# Autodesk Inventor assembly: CardGuideArray-Long
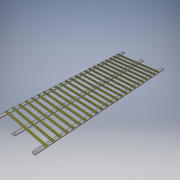
[picture p0: Inventor's stored thumbnail of the model, 180x180]
Saved by Autodesk Inventor 2018 (Build 220112000, 112)
## iProperties
Created: 2025-02-19
Part Number: CardGuideArray-Long
Material: Všeobecné
Document SubType Name: Assembly
Designer: Jozko Mrkvicka
Author: Jozko Mrkvicka
## Documents named in this file (5)
- D:\05_Projekty\Projects_Inventor\Haluska9000\CardGuideArray-8-Inch.iam
- D:\05_Projekty\Projects_Inventor\Haluska9000\CardGuide.ipt
- D:\05_Projekty\Projects_Inventor\Haluska9000\Profile-Flat.ipt
- D:\05_Projekty\Projects_Inventor\Haluska9000\Profile-Flat\Profile-Flat#Cabinet-FerriteCore-Width.ipt
- D:\05_Projekty\Projects_Inventor\Haluska9000\CardGuide\CardGuide#8-inch.ipt
## Components (26 placed, 2 different names)
1. Profile-Flat#Cabinet-FerriteCore-Width:3 — Stejný směr:3, Stejný směr:4, Proti sobě:93, Proti sobě:94, Proti sobě:95, Proti sobě:96, Proti sobě:97, Proti sobě:98, Proti sobě:99, Proti sobě:100, Proti sobě:101, Proti sobě:102, Proti sobě:114, Proti sobě:115, Proti sobě:116, Proti sobě:117, Proti sobě:118, Proti sobě:119, Proti sobě:120, Proti sobě:121, Proti sobě:122, Proti sobě:123, Proti sobě:124, Proti sobě:125, Proti sobě:126, Proti sobě:127, Proti sobě:128, Proti sobě:129, Proti sobě:130, Proti sobě:131, Proti sobě:132, Proti sobě:133, Proti sobě:134, Proti sobě:135, Proti sobě:136
2. Profile-Flat#Cabinet-FerriteCore-Width:4 — Proti sobě:42, Proti sobě:43, Proti sobě:44, Proti sobě:45, Proti sobě:46, Proti sobě:47, Proti sobě:48, Proti sobě:49, Proti sobě:50, Proti sobě:51, Proti sobě:52, Proti sobě:53, Proti sobě:54, Proti sobě:55, Proti sobě:56, Proti sobě:57, Proti sobě:58, Proti sobě:59, Proti sobě:60, Proti sobě:61, Proti sobě:62, Proti sobě:63, Proti sobě:64, Proti sobě:65, Proti sobě:66, Proti sobě:67, Stejný směr:3, Stejný směr:4, Stejný směr:5, Proti sobě:103, Proti sobě:104, Proti sobě:105, Proti sobě:106, Proti sobě:107, Proti sobě:108, Proti sobě:109, Proti sobě:110, Proti sobě:111, Proti sobě:112, Proti sobě:113
3. Profile-Flat#Cabinet-FerriteCore-Width:5 — Stejný směr:5
4. CardGuide#8-inch:14 — Proti sobě:45, Proti sobě:64, Proti sobě:129
5. CardGuide#8-inch:15 — Proti sobě:46, Proti sobě:63, Proti sobě:128
6. CardGuide#8-inch:16 — Proti sobě:54, Proti sobě:55, Proti sobě:119
7. CardGuide#8-inch:17 — Proti sobě:44, Proti sobě:65, Proti sobě:130
8. CardGuide#8-inch:18 — Proti sobě:47, Proti sobě:62, Proti sobě:127
9. CardGuide#8-inch:19 — Proti sobě:48, Proti sobě:61, Proti sobě:126
10. CardGuide#8-inch:20 — Proti sobě:42, Proti sobě:67, Proti sobě:120
11. CardGuide#8-inch:21 — Proti sobě:43, Proti sobě:66, Proti sobě:131
12. CardGuide#8-inch:22 — Proti sobě:50, Proti sobě:59, Proti sobě:124
13. CardGuide#8-inch:23 — Proti sobě:51, Proti sobě:58, Proti sobě:123
14. CardGuide#8-inch:24 — Proti sobě:52, Proti sobě:57, Proti sobě:122
15. CardGuide#8-inch:25 — Proti sobě:53, Proti sobě:56, Proti sobě:121
16. CardGuide#8-inch:26 — Proti sobě:49, Proti sobě:60, Proti sobě:125
17. CardGuide#8-inch:27 — Proti sobě:95, Proti sobě:105, Proti sobě:134
18. CardGuide#8-inch:28 — Proti sobě:96, Proti sobě:104, Proti sobě:133
19. CardGuide#8-inch:29 — Proti sobě:94, Proti sobě:106, Proti sobě:135
20. CardGuide#8-inch:30 — Proti sobě:97, Proti sobě:103, Proti sobě:132
21. CardGuide#8-inch:31 — Proti sobě:93, Proti sobě:107, Proti sobě:136
22. CardGuide#8-inch:32 — Proti sobě:100, Proti sobě:110, Proti sobě:116
23. CardGuide#8-inch:33 — Proti sobě:101, Proti sobě:111, Proti sobě:115
24. CardGuide#8-inch:34 — Proti sobě:99, Proti sobě:109, Proti sobě:117
25. CardGuide#8-inch:35 — Proti sobě:102, Proti sobě:112, Proti sobě:114
26. CardGuide#8-inch:36 — Proti sobě:98, Proti sobě:108, Proti sobě:118
## Relationships (73: Mate 70, Flush 3)
- Proti sobě:42 [Mate]: Profile-Flat#Cabinet-FerriteCore-Width:4 ↔ CardGuide#8-inch:20
- Proti sobě:43 [Mate]: Profile-Flat#Cabinet-FerriteCore-Width:4 ↔ CardGuide#8-inch:21
- Proti sobě:44 [Mate]: Profile-Flat#Cabinet-FerriteCore-Width:4 ↔ CardGuide#8-inch:17
- Proti sobě:45 [Mate]: Profile-Flat#Cabinet-FerriteCore-Width:4 ↔ CardGuide#8-inch:14
- Proti sobě:46 [Mate]: Profile-Flat#Cabinet-FerriteCore-Width:4 ↔ CardGuide#8-inch:15
- Proti sobě:47 [Mate]: Profile-Flat#Cabinet-FerriteCore-Width:4 ↔ CardGuide#8-inch:18
- Proti sobě:48 [Mate]: Profile-Flat#Cabinet-FerriteCore-Width:4 ↔ CardGuide#8-inch:19
- Proti sobě:49 [Mate]: Profile-Flat#Cabinet-FerriteCore-Width:4 ↔ CardGuide#8-inch:26
- Proti sobě:50 [Mate]: Profile-Flat#Cabinet-FerriteCore-Width:4 ↔ CardGuide#8-inch:22
- Proti sobě:51 [Mate]: Profile-Flat#Cabinet-FerriteCore-Width:4 ↔ CardGuide#8-inch:23
- Proti sobě:52 [Mate]: Profile-Flat#Cabinet-FerriteCore-Width:4 ↔ CardGuide#8-inch:24
- Proti sobě:53 [Mate]: Profile-Flat#Cabinet-FerriteCore-Width:4 ↔ CardGuide#8-inch:25
- Proti sobě:54 [Mate]: Profile-Flat#Cabinet-FerriteCore-Width:4 ↔ CardGuide#8-inch:16
- Proti sobě:55 [Mate]: Profile-Flat#Cabinet-FerriteCore-Width:4 ↔ CardGuide#8-inch:16
- Proti sobě:56 [Mate]: Profile-Flat#Cabinet-FerriteCore-Width:4 ↔ CardGuide#8-inch:25
- Proti sobě:57 [Mate]: Profile-Flat#Cabinet-FerriteCore-Width:4 ↔ CardGuide#8-inch:24
- Proti sobě:58 [Mate]: Profile-Flat#Cabinet-FerriteCore-Width:4 ↔ CardGuide#8-inch:23
- Proti sobě:59 [Mate]: Profile-Flat#Cabinet-FerriteCore-Width:4 ↔ CardGuide#8-inch:22
- Proti sobě:60 [Mate]: Profile-Flat#Cabinet-FerriteCore-Width:4 ↔ CardGuide#8-inch:26
- Proti sobě:61 [Mate]: Profile-Flat#Cabinet-FerriteCore-Width:4 ↔ CardGuide#8-inch:19
- Proti sobě:62 [Mate]: Profile-Flat#Cabinet-FerriteCore-Width:4 ↔ CardGuide#8-inch:18
- Proti sobě:63 [Mate]: Profile-Flat#Cabinet-FerriteCore-Width:4 ↔ CardGuide#8-inch:15
- Proti sobě:64 [Mate]: Profile-Flat#Cabinet-FerriteCore-Width:4 ↔ CardGuide#8-inch:14
- Proti sobě:65 [Mate]: Profile-Flat#Cabinet-FerriteCore-Width:4 ↔ CardGuide#8-inch:17
- Proti sobě:66 [Mate]: Profile-Flat#Cabinet-FerriteCore-Width:4 ↔ CardGuide#8-inch:21
- Proti sobě:67 [Mate]: Profile-Flat#Cabinet-FerriteCore-Width:4 ↔ CardGuide#8-inch:20
- Stejný směr:3 [Flush]: Profile-Flat#Cabinet-FerriteCore-Width:3 ↔ Profile-Flat#Cabinet-FerriteCore-Width:4
- Stejný směr:4 [Flush]: Profile-Flat#Cabinet-FerriteCore-Width:3 ↔ Profile-Flat#Cabinet-FerriteCore-Width:4
- Stejný směr:5 [Flush]: Profile-Flat#Cabinet-FerriteCore-Width:4 ↔ Profile-Flat#Cabinet-FerriteCore-Width:5
- Proti sobě:93 [Mate]: Profile-Flat#Cabinet-FerriteCore-Width:3 ↔ CardGuide#8-inch:31
- Proti sobě:94 [Mate]: Profile-Flat#Cabinet-FerriteCore-Width:3 ↔ CardGuide#8-inch:29
- Proti sobě:95 [Mate]: Profile-Flat#Cabinet-FerriteCore-Width:3 ↔ CardGuide#8-inch:27
- Proti sobě:96 [Mate]: Profile-Flat#Cabinet-FerriteCore-Width:3 ↔ CardGuide#8-inch:28
- Proti sobě:97 [Mate]: Profile-Flat#Cabinet-FerriteCore-Width:3 ↔ CardGuide#8-inch:30
- Proti sobě:98 [Mate]: Profile-Flat#Cabinet-FerriteCore-Width:3 ↔ CardGuide#8-inch:36
- Proti sobě:99 [Mate]: Profile-Flat#Cabinet-FerriteCore-Width:3 ↔ CardGuide#8-inch:34
- Proti sobě:100 [Mate]: Profile-Flat#Cabinet-FerriteCore-Width:3 ↔ CardGuide#8-inch:32
- Proti sobě:101 [Mate]: Profile-Flat#Cabinet-FerriteCore-Width:3 ↔ CardGuide#8-inch:33
- Proti sobě:102 [Mate]: Profile-Flat#Cabinet-FerriteCore-Width:3 ↔ CardGuide#8-inch:35
- Proti sobě:103 [Mate]: Profile-Flat#Cabinet-FerriteCore-Width:4 ↔ CardGuide#8-inch:30
- Proti sobě:104 [Mate]: Profile-Flat#Cabinet-FerriteCore-Width:4 ↔ CardGuide#8-inch:28
- Proti sobě:105 [Mate]: Profile-Flat#Cabinet-FerriteCore-Width:4 ↔ CardGuide#8-inch:27
- Proti sobě:106 [Mate]: Profile-Flat#Cabinet-FerriteCore-Width:4 ↔ CardGuide#8-inch:29
- Proti sobě:107 [Mate]: Profile-Flat#Cabinet-FerriteCore-Width:4 ↔ CardGuide#8-inch:31
- Proti sobě:108 [Mate]: Profile-Flat#Cabinet-FerriteCore-Width:4 ↔ CardGuide#8-inch:36
- Proti sobě:109 [Mate]: Profile-Flat#Cabinet-FerriteCore-Width:4 ↔ CardGuide#8-inch:34
- Proti sobě:110 [Mate]: Profile-Flat#Cabinet-FerriteCore-Width:4 ↔ CardGuide#8-inch:32
- Proti sobě:111 [Mate]: Profile-Flat#Cabinet-FerriteCore-Width:4 ↔ CardGuide#8-inch:33
- Proti sobě:112 [Mate]: Profile-Flat#Cabinet-FerriteCore-Width:4 ↔ CardGuide#8-inch:35
- Proti sobě:113 [Mate]: Profile-Flat#Cabinet-FerriteCore-Width:4
- Proti sobě:114 [Mate]: Profile-Flat#Cabinet-FerriteCore-Width:3 ↔ CardGuide#8-inch:35
- Proti sobě:115 [Mate]: Profile-Flat#Cabinet-FerriteCore-Width:3 ↔ CardGuide#8-inch:33
- Proti sobě:116 [Mate]: Profile-Flat#Cabinet-FerriteCore-Width:3 ↔ CardGuide#8-inch:32
- Proti sobě:117 [Mate]: Profile-Flat#Cabinet-FerriteCore-Width:3 ↔ CardGuide#8-inch:34
- Proti sobě:118 [Mate]: Profile-Flat#Cabinet-FerriteCore-Width:3 ↔ CardGuide#8-inch:36
- Proti sobě:119 [Mate]: Profile-Flat#Cabinet-FerriteCore-Width:3 ↔ CardGuide#8-inch:16
- Proti sobě:120 [Mate]: Profile-Flat#Cabinet-FerriteCore-Width:3 ↔ CardGuide#8-inch:20
- Proti sobě:121 [Mate]: Profile-Flat#Cabinet-FerriteCore-Width:3 ↔ CardGuide#8-inch:25
- Proti sobě:122 [Mate]: Profile-Flat#Cabinet-FerriteCore-Width:3 ↔ CardGuide#8-inch:24
- Proti sobě:123 [Mate]: Profile-Flat#Cabinet-FerriteCore-Width:3 ↔ CardGuide#8-inch:23
- Proti sobě:124 [Mate]: Profile-Flat#Cabinet-FerriteCore-Width:3 ↔ CardGuide#8-inch:22
- Proti sobě:125 [Mate]: Profile-Flat#Cabinet-FerriteCore-Width:3 ↔ CardGuide#8-inch:26
- Proti sobě:126 [Mate]: Profile-Flat#Cabinet-FerriteCore-Width:3 ↔ CardGuide#8-inch:19
- Proti sobě:127 [Mate]: Profile-Flat#Cabinet-FerriteCore-Width:3 ↔ CardGuide#8-inch:18
- Proti sobě:128 [Mate]: Profile-Flat#Cabinet-FerriteCore-Width:3 ↔ CardGuide#8-inch:15
- Proti sobě:129 [Mate]: Profile-Flat#Cabinet-FerriteCore-Width:3 ↔ CardGuide#8-inch:14
- Proti sobě:130 [Mate]: Profile-Flat#Cabinet-FerriteCore-Width:3 ↔ CardGuide#8-inch:17
- Proti sobě:131 [Mate]: Profile-Flat#Cabinet-FerriteCore-Width:3 ↔ CardGuide#8-inch:21
- Proti sobě:132 [Mate]: Profile-Flat#Cabinet-FerriteCore-Width:3 ↔ CardGuide#8-inch:30
- Proti sobě:133 [Mate]: Profile-Flat#Cabinet-FerriteCore-Width:3 ↔ CardGuide#8-inch:28
- Proti sobě:134 [Mate]: Profile-Flat#Cabinet-FerriteCore-Width:3 ↔ CardGuide#8-inch:27
- Proti sobě:135 [Mate]: Profile-Flat#Cabinet-FerriteCore-Width:3 ↔ CardGuide#8-inch:29
- Proti sobě:136 [Mate]: Profile-Flat#Cabinet-FerriteCore-Width:3 ↔ CardGuide#8-inch:31
